# Autodesk Inventor assembly: Gripper
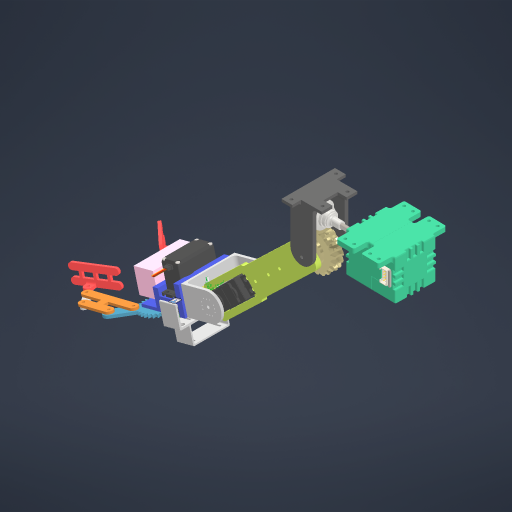
[picture p0: Inventor's stored thumbnail of the model, 512x512]
Saved by Autodesk Inventor 2023.1 (Build 271208000, 208)
## iProperties
Created: 2022-10-21
Part Number: Gripper
Document SubType Name: Assembly
Designer: amtat
Author: amtat
## Documents named in this file (22)
- C:\Users\amtat\OneDrive - uc.cl\UC\Año 5\Sem 2\Capstone\Gripper\Gripper.iam
- C:\Users\amtat\OneDrive - uc.cl\UC\Año 5\Sem 2\Capstone\Gripper\g1k.ipt
- C:\Users\amtat\OneDrive - uc.cl\UC\Año 5\Sem 2\Capstone\Gripper\TOWER PRO MG-995, ANALOG SERVO v9.iam
- C:\Users\amtat\OneDrive - uc.cl\UC\Año 5\Sem 2\Capstone\Gripper\dd3y.ipt
- C:\Users\amtat\OneDrive - uc.cl\UC\Año 5\Sem 2\Capstone\Gripper\antebrazo.ipt
- C:\Users\amtat\OneDrive - uc.cl\UC\Año 5\Sem 2\Capstone\Gripper\acople_1.ipt
- C:\Users\amtat\OneDrive - uc.cl\UC\Año 5\Sem 2\Capstone\Gripper\engranaje_acr.ipt
- C:\Users\amtat\OneDrive - uc.cl\UC\Año 5\Sem 2\Capstone\Gripper\acople_acr.ipt
- C:\Users\amtat\OneDrive - uc.cl\UC\Año 5\Sem 2\Capstone\Gripper\union_acr.ipt
- C:\Users\amtat\OneDrive - uc.cl\UC\Año 5\Sem 2\Capstone\Gripper\acople_gripper.ipt
- C:\Users\amtat\OneDrive - uc.cl\UC\Año 5\Sem 2\Capstone\Gripper\agarre_derecha.ipt
- C:\Users\amtat\OneDrive - uc.cl\UC\Año 5\Sem 2\Capstone\Gripper\agarre_izquierda.ipt
- C:\Users\amtat\OneDrive - uc.cl\UC\Año 5\Sem 2\Capstone\Gripper\acople_2.ipt
- C:\Users\amtat\OneDrive - uc.cl\UC\Año 5\Sem 2\Capstone\Gripper\soporte_sensor.ipt
- C:\Users\amtat\OneDrive - uc.cl\UC\Año 5\Sem 2\Capstone\Gripper\Ultra Sonic Sensor.ipt
- C:\Users\amtat\OneDrive - uc.cl\UC\Año 5\Sem 2\Capstone\Gripper\Nema.ipt
- C:\Users\amtat\OneDrive - uc.cl\UC\Año 5\Sem 2\Capstone\Gripper\NEMA_top_case.ipt
- C:\Users\amtat\OneDrive - uc.cl\UC\Año 5\Sem 2\Capstone\Gripper\NEMA_bottom_case.ipt
- C:\Users\amtat\OneDrive - uc.cl\UC\Año 5\Sem 2\Capstone\Gripper\Worm1.ipt
- C:\Users\amtat\OneDrive - uc.cl\UC\Año 5\Sem 2\Capstone\Gripper\Worm Gear1.ipt
- C:\Users\amtat\OneDrive - uc.cl\UC\Año 5\Sem 2\Capstone\Gripper\soporte_brazo.ipt
- C:\Users\amtat\OneDrive - uc.cl\UC\Año 5\Sem 2\Capstone\Gripper\soporte_camara.ipt
## Components (25 placed, 21 different names)
1. g1k:1 — Insert:1, Insert:2, Insert:9, Insert:10, Insert:12, Insert:13, Insert:28, Insert:29, Insert:42
2. TOWER PRO MG-995, ANALOG SERVO v9:1 [sub-assembly] — Insert:1, Insert:2, Insert:3
3. dd3y:1 — Insert:3
4. antebrazo:1 — Insert:4, Insert:5, Rotation:1, Insert:26, Insert:27, Insert:39, Insert:40, Insert:41
5. TOWER PRO MG-995, ANALOG SERVO v9:2 [sub-assembly] — Insert:4, Insert:5, Insert:8, Insert:11
6. acople_1:1 — Insert:8, Insert:9, Insert:10, Rotation:1, Insert:11
7. engranaje_acr:1 — Insert:12, Insert:14, Insert:15, Insert:19
8. engranaje_acr:2 — Insert:13, Insert:16, Insert:17, Insert:18
9. acople_acr:1 — Insert:14, Insert:15, Insert:21, Insert:23
10. acople_acr:2 — Insert:16, Insert:17, Insert:20, Insert:22
11. union_acr:1 — Insert:18, Insert:19
12. acople_gripper:1 — Insert:20, Insert:22, Insert:24
13. acople_gripper:2 — Insert:21, Insert:23, Insert:25
14. agarre_derecha:1 — Insert:24
15. agarre_izquierda:1 — Insert:25
16. acople_2:1 — Insert:26, Insert:27
17. soporte_sensor:1 — Insert:28, Insert:29, Mate:1, Mate:2, Flush:1
18. Ultra Sonic Sensor:1 — Mate:1, Mate:2, Flush:1
19. Nema:1 — Insert:36, Insert:37, Insert:38
20. NEMA_top_case:1 — Insert:36, Insert:37, Flush:2, Flush:3, Mate:3, Flush:4
21. NEMA_bottom_case:1 — Flush:2, Flush:3, Mate:3
22. Worm:1 — Insert:38
23. Worm Gear:1 — Insert:39, Insert:40
24. soporte_brazo:1 — Insert:41, Flush:4
25. soporte_camara:1 — Insert:42
## Relationships (42: Insert 34, Flush 4, Mate 3, RelateRotation 1)
- Insert:1: g1k:1 ↔ TOWER PRO MG-995, ANALOG SERVO v9:1
- Insert:2: g1k:1 ↔ TOWER PRO MG-995, ANALOG SERVO v9:1
- Insert:3: TOWER PRO MG-995, ANALOG SERVO v9:1 ↔ dd3y:1
- Insert:4: antebrazo:1 ↔ TOWER PRO MG-995, ANALOG SERVO v9:2
- Insert:5: antebrazo:1 ↔ TOWER PRO MG-995, ANALOG SERVO v9:2
- Insert:8: TOWER PRO MG-995, ANALOG SERVO v9:2 ↔ acople_1:1
- Insert:9: g1k:1 ↔ acople_1:1
- Insert:10: g1k:1 ↔ acople_1:1
- Rotation:1 [RelateRotation] (1 ul): antebrazo:1 ↔ acople_1:1
- Insert:11: TOWER PRO MG-995, ANALOG SERVO v9:2 ↔ acople_1:1
- Insert:12: g1k:1 ↔ engranaje_acr:1
- Insert:13: g1k:1 ↔ engranaje_acr:2
- Insert:14: engranaje_acr:1 ↔ acople_acr:1
- Insert:15: engranaje_acr:1 ↔ acople_acr:1
- Insert:16: engranaje_acr:2 ↔ acople_acr:2
- Insert:17: engranaje_acr:2 ↔ acople_acr:2
- Insert:18: engranaje_acr:2 ↔ union_acr:1
- Insert:19: engranaje_acr:1 ↔ union_acr:1
- Insert:20: acople_acr:2 ↔ acople_gripper:1
- Insert:21: acople_acr:1 ↔ acople_gripper:2
- Insert:22: acople_acr:2 ↔ acople_gripper:1
- Insert:23: acople_acr:1 ↔ acople_gripper:2
- Insert:24: acople_gripper:1 ↔ agarre_derecha:1
- Insert:25: acople_gripper:2 ↔ agarre_izquierda:1
- Insert:26: antebrazo:1 ↔ acople_2:1
- Insert:27: antebrazo:1 ↔ acople_2:1
- Insert:28: g1k:1 ↔ soporte_sensor:1
- Insert:29: g1k:1 ↔ soporte_sensor:1
- Mate:1 (0.15 mm): soporte_sensor:1 ↔ Ultra Sonic Sensor:1
- Mate:2 (1.75 mm): soporte_sensor:1 ↔ Ultra Sonic Sensor:1
- Flush:1 (2 mm): soporte_sensor:1 ↔ Ultra Sonic Sensor:1
- Insert:36: Nema:1 ↔ NEMA_top_case:1
- Insert:37: Nema:1 ↔ NEMA_top_case:1
- Flush:2: NEMA_top_case:1 ↔ NEMA_bottom_case:1
- Flush:3: NEMA_top_case:1 ↔ NEMA_bottom_case:1
- Mate:3: NEMA_top_case:1 ↔ NEMA_bottom_case:1
- Insert:38: Nema:1 ↔ Worm:1
- Insert:39: antebrazo:1 ↔ Worm Gear:1
- Insert:40: antebrazo:1 ↔ Worm Gear:1
- Insert:41: antebrazo:1 ↔ soporte_brazo:1
- Flush:4: NEMA_top_case:1 ↔ soporte_brazo:1
- Insert:42: g1k:1 ↔ soporte_camara:1
